# Autodesk Inventor assembly: ROBOT_1_3
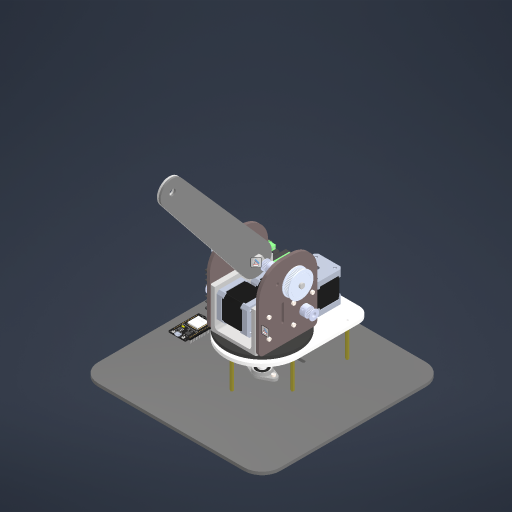
[picture p0: Inventor's stored thumbnail of the model, 512x512]
Saved by Autodesk Inventor 2023 (Build 270158000, 158)
## iProperties
Created: 2023-09-06
Part Number: ROBOT_1_3
Document SubType Name: Assembly
Designer: philo
Sending System: Autodesk Inventor 2023
Preprocessor: ST-DEVELOPER v19
Title: C:\Users\philo\OneDrive\Desktop\HK1-2024\TT ROBOT\3DVer2\ROBOT_1_2.stp
Author: philo
## Documents named in this file (25)
- C:\Users\philo\OneDrive\Desktop\HK1-2024\TT ROBOT\02_3D_design\ROBOT_1_3.iam
- C:\Users\philo\OneDrive\Desktop\HK1-2024\TT ROBOT\02_3D_design\DeRobot.ipt
- C:\Users\philo\OneDrive\Desktop\HK1-2024\TT ROBOT\02_3D_design\Detron.ipt
- C:\Users\philo\OneDrive\Desktop\HK1-2024\TT ROBOT\02_3D_design\goidoObi.ipt
- C:\Users\philo\OneDrive\Desktop\HK1-2024\TT ROBOT\02_3D_design\truday.ipt
- C:\Users\philo\OneDrive\Desktop\HK1-2024\TT ROBOT\02_3D_design\gt2_60teeth.iam
- C:\Users\philo\OneDrive\Desktop\HK1-2024\TT ROBOT\02_3D_design\STEP MOTOR NEMA 17.ipt
- C:\Users\philo\OneDrive\Desktop\HK1-2024\TT ROBOT\02_3D_design\GT2 Pulley 20 Tooth (ID6mm).ipt
- C:\Users\philo\OneDrive\Desktop\HK1-2024\TT ROBOT\02_3D_design\M3 x 5mm.ipt
- C:\Users\philo\OneDrive\Desktop\HK1-2024\TT ROBOT\02_3D_design\Diaquay.ipt
- C:\Users\philo\OneDrive\Desktop\HK1-2024\TT ROBOT\02_3D_design\Tb6600.ipt
- C:\Users\philo\OneDrive\Desktop\HK1-2024\TT ROBOT\02_3D_design\ESP-WROOM32.iam
- C:\Users\philo\OneDrive\Desktop\HK1-2024\TT ROBOT\02_3D_design\codinhtruc.ipt
- C:\Users\philo\OneDrive\Desktop\HK1-2024\TT ROBOT\02_3D_design\daydai.ipt
- C:\Users\philo\OneDrive\Desktop\HK1-2024\TT ROBOT\02_3D_design\gt2smooth.ipt
- C:\Users\philo\OneDrive\Desktop\HK1-2024\TT ROBOT\02_3D_design\trudong5mm.ipt
- C:\Users\philo\OneDrive\Desktop\HK1-2024\TT ROBOT\02_3D_design\trucdogt2.ipt
- C:\Users\philo\OneDrive\Desktop\HK1-2024\TT ROBOT\02_3D_design\HALL.ipt
- C:\Users\philo\OneDrive\Desktop\HK1-2024\TT ROBOT\02_3D_design\namcham.ipt
- C:\Users\philo\OneDrive\Desktop\HK1-2024\TT ROBOT\02_3D_design\Tamop1.ipt
- C:\Users\philo\OneDrive\Desktop\HK1-2024\TT ROBOT\02_3D_design\60pitch pulley GT2 6mm ASSEMBLY.iam
- C:\Users\philo\OneDrive\Desktop\HK1-2024\TT ROBOT\02_3D_design\truc8mm.ipt
- C:\Users\philo\OneDrive\Desktop\HK1-2024\TT ROBOT\02_3D_design\giulink2.ipt
- C:\Users\philo\OneDrive\Documents\Link2Base.ipt
- C:\Users\philo\OneDrive\Desktop\HK1-2024\TT ROBOT\02_3D_design\OcM8.ipt
## Components (61 placed, 24 different names)
1. GT2 Pulley 20 Tooth (ID6mm):4 — Mate:73, Flush:8
2. Link2Base:2 — Mate:74, Mate:75, Mate:76, Mate:78
3. OcM8:1 — Mate:77, Flush:9, Mate:78
4. OcM8:2 — Mate:79, Mate:80
5. DeRobot:1 — Angle:9
6. Detron:1 — Mate:33
7. goidoObi:1
8. goidoObi:2
9. truday:1 — Mate:32
10. gt2_60teeth:1 [sub-assembly]
11. STEP MOTOR NEMA 17:1
12. GT2 Pulley 20 Tooth (ID6mm):1
13. M3 x 5mm:1
14. M3 x 5mm:2
15. M3 x 5mm:3
16. M3 x 5mm:5
17. M3 x 5mm:6
18. M3 x 5mm:7
19. M3 x 5mm:8
20. Tb6600:1
21. Tb6600:2
22. ESP-WROOM32:1 [sub-assembly]
23. daydai:1
24. gt2smooth:1
25. trudong5mm:4
26. trudong5mm:5
27. trudong5mm:6
28. trudong5mm:8
29. trudong5mm:9
30. trucdogt2:1
31. HALL:1
32. M3 x 5mm:9 — Mate:38, Mate:56
33. M3 x 5mm:10 — Mate:39, Mate:58
34. M3 x 5mm:11 — Mate:37, Mate:60
35. M3 x 5mm:12 — Mate:40, Mate:57
36. M3 x 5mm:13 — Mate:41, Mate:61
37. M3 x 5mm:14 — Mate:42, Mate:59
38. M3 x 5mm:15 — Mate:43, Mate:52
39. M3 x 5mm:16 — Mate:45, Mate:51
40. M3 x 5mm:17 — Mate:46, Mate:54
41. M3 x 5mm:18 — Mate:44, Mate:50
42. M3 x 5mm:19 — Mate:47, Mate:53
43. M3 x 5mm:20 — Mate:48, Mate:55
44. gt2smooth:2 — Mate:49
45. giulink2:1 — Mate:63, Angle:3, Angle:4, Angle:5, Angle:6, Angle:7, Angle:8, Mate:64, Mate:65, Mate:67, Flush:4, Flush:5, Mate:68, Mate:69
46. Diaquay:1 — Mate:1, Mate:2, Mate:7, Mate:8, Mate:32, Mate:33, Mate:34, Angle:1, Angle:2, Flush:2, Mate:62, Flush:3, Angle:7
47. codinhtruc:2 — Mate:1, Mate:2, Mate:34, Mate:63
48. namcham:1 — Angle:2, Flush:2, Mate:62, Flush:3
49. STEP MOTOR NEMA 17:2 — Mate:27, Mate:28, Angle:6, Mate:66, Mate:67
50. STEP MOTOR NEMA 17:3 — Mate:26, Mate:30, Angle:5, Angle:8, Mate:64, Mate:65
51. Tamop1:1 — Mate:7, Mate:11, Mate:14, Mate:15, Mate:21, Flush:1, Mate:27, Mate:29, Mate:37, Mate:38, Mate:39, Mate:40, Mate:41, Mate:42, Mate:56, Mate:57, Mate:58, Mate:59, Mate:60, Mate:61, Angle:3, Mate:66, Flush:4, Mate:69, Angle:9
52. goidoObi:3 — Mate:11, Mate:14, Mate:15, Mate:18
53. GT2 Pulley 20 Tooth (ID6mm):2 — Mate:28, Mate:29
54. 60pitch pulley GT2 6mm ASSEMBLY:1 [sub-assembly] — Mate:21, Mate:22
55. Tamop1:2 — Mate:8, Mate:12, Mate:13, Mate:16, Mate:19, Mate:26, Mate:31, Angle:1, Mate:43, Mate:44, Mate:45, Mate:46, Mate:47, Mate:48, Mate:49, Mate:50, Mate:51, Mate:52, Mate:53, Mate:54, Mate:55, Angle:4, Flush:5, Mate:68, Angle:10
56. goidoObi:4 — Mate:12, Mate:13, Mate:16, Mate:17
57. GT2 Pulley 20 Tooth (ID6mm):3 — Mate:30, Mate:31
58. 60pitch pulley GT2 6mm ASSEMBLY:2 [sub-assembly] — Mate:19, Mate:20
59. truc8mm:1 — Mate:18, Mate:22, Mate:23, Flush:1, Mate:73, Flush:8
60. truc8mm:2 — Mate:17, Mate:20, Mate:23, Mate:70, Mate:74, Mate:77, Flush:9, Mate:79
61. Link2Base:1 — Mate:70, Angle:10, Mate:75, Mate:76, Mate:80
## Relationships (85: Mate 68, Angle 10, Flush 7)
- Mate:1: Diaquay:1 ↔ codinhtruc:2
- Mate:2: Diaquay:1 ↔ codinhtruc:2
- Mate:7: Diaquay:1 ↔ Tamop1:1
- Mate:8: Diaquay:1 ↔ Tamop1:2
- Mate:11: Tamop1:1 ↔ goidoObi:3
- Mate:12: Tamop1:2 ↔ goidoObi:4
- Mate:13: Tamop1:2 ↔ goidoObi:4
- Mate:14: Tamop1:1 ↔ goidoObi:3
- Mate:15: Tamop1:1 ↔ goidoObi:3
- Mate:16: Tamop1:2 ↔ goidoObi:4
- Mate:17: goidoObi:4 ↔ truc8mm:2
- Mate:18: goidoObi:3 ↔ truc8mm:1
- Mate:19 (3 mm): Tamop1:2 ↔ 60pitch pulley GT2 6mm ASSEMBLY:2
- Mate:20: 60pitch pulley GT2 6mm ASSEMBLY:2 ↔ truc8mm:2
- Mate:21 (3 mm): Tamop1:1 ↔ 60pitch pulley GT2 6mm ASSEMBLY:1
- Mate:22: 60pitch pulley GT2 6mm ASSEMBLY:1 ↔ truc8mm:1
- Mate:23 (5 mm): truc8mm:1 ↔ truc8mm:2
- Flush:1 (-36 mm): Tamop1:1 ↔ truc8mm:1
- Mate:26: STEP MOTOR NEMA 17:3 ↔ Tamop1:2
- Mate:27: STEP MOTOR NEMA 17:2 ↔ Tamop1:1
- Mate:28: STEP MOTOR NEMA 17:2 ↔ GT2 Pulley 20 Tooth (ID6mm):2
- Mate:29 (3 mm): Tamop1:1 ↔ GT2 Pulley 20 Tooth (ID6mm):2
- Mate:30: STEP MOTOR NEMA 17:3 ↔ GT2 Pulley 20 Tooth (ID6mm):3
- Mate:31 (3 mm): Tamop1:2 ↔ GT2 Pulley 20 Tooth (ID6mm):3
- Mate:32: truday:1 ↔ Diaquay:1
- Mate:33 (6 mm): Detron:1 ↔ Diaquay:1
- Mate:34: Diaquay:1 ↔ codinhtruc:2
- Angle:1 (0 deg): Diaquay:1 ↔ Tamop1:2
- Angle:2 (0 deg): Diaquay:1 ↔ namcham:1
- Flush:2 (-60 mm): Diaquay:1 ↔ namcham:1
- Mate:37: M3 x 5mm:11 ↔ Tamop1:1
- Mate:38: M3 x 5mm:9 ↔ Tamop1:1
- Mate:39: M3 x 5mm:10 ↔ Tamop1:1
- Mate:40: M3 x 5mm:12 ↔ Tamop1:1
- Mate:41: M3 x 5mm:13 ↔ Tamop1:1
- Mate:42: M3 x 5mm:14 ↔ Tamop1:1
- Mate:43: M3 x 5mm:15 ↔ Tamop1:2
- Mate:44: M3 x 5mm:18 ↔ Tamop1:2
- Mate:45: M3 x 5mm:16 ↔ Tamop1:2
- Mate:46: M3 x 5mm:17 ↔ Tamop1:2
- Mate:47: M3 x 5mm:19 ↔ Tamop1:2
- Mate:48: M3 x 5mm:20 ↔ Tamop1:2
- Mate:49 (8 mm): gt2smooth:2 ↔ Tamop1:2
- Mate:50: M3 x 5mm:18 ↔ Tamop1:2
- Mate:51: M3 x 5mm:16 ↔ Tamop1:2
- Mate:52: M3 x 5mm:15 ↔ Tamop1:2
- Mate:53: M3 x 5mm:19 ↔ Tamop1:2
- Mate:54: M3 x 5mm:17 ↔ Tamop1:2
- Mate:55: M3 x 5mm:20 ↔ Tamop1:2
- Mate:56: M3 x 5mm:9 ↔ Tamop1:1
- Mate:57: M3 x 5mm:12 ↔ Tamop1:1
- Mate:58: M3 x 5mm:10 ↔ Tamop1:1
- Mate:59: M3 x 5mm:14 ↔ Tamop1:1
- Mate:60: M3 x 5mm:11 ↔ Tamop1:1
- Mate:61: M3 x 5mm:13 ↔ Tamop1:1
- Mate:62 (-3 mm): Diaquay:1 ↔ namcham:1
- Flush:3: Diaquay:1 ↔ namcham:1
- Mate:63: giulink2:1 ↔ codinhtruc:2
- Angle:3 (90 deg): giulink2:1 ↔ Tamop1:1
- Angle:4 (90 deg): giulink2:1 ↔ Tamop1:2
- Angle:5 (0 deg): giulink2:1 ↔ STEP MOTOR NEMA 17:3
- Angle:6 (0 deg): giulink2:1 ↔ STEP MOTOR NEMA 17:2
- Angle:7 (90 deg): giulink2:1 ↔ Diaquay:1
- Angle:8 (0 deg): giulink2:1 ↔ STEP MOTOR NEMA 17:3
- Mate:64: giulink2:1 ↔ STEP MOTOR NEMA 17:3
- Mate:65: giulink2:1 ↔ STEP MOTOR NEMA 17:3
- Mate:66: STEP MOTOR NEMA 17:2 ↔ Tamop1:1
- Mate:67: giulink2:1 ↔ STEP MOTOR NEMA 17:2
- Flush:4: giulink2:1 ↔ Tamop1:1
- Flush:5: giulink2:1 ↔ Tamop1:2
- Mate:68: giulink2:1 ↔ Tamop1:2
- Mate:69: giulink2:1 ↔ Tamop1:1
- Angle:9 (0 deg): DeRobot:1 ↔ Tamop1:1
- Mate:70: truc8mm:2 ↔ Link2Base:1
- Mate:73: GT2 Pulley 20 Tooth (ID6mm):4 ↔ truc8mm:1
- Flush:8 (3 mm): GT2 Pulley 20 Tooth (ID6mm):4 ↔ truc8mm:1
- Angle:10 (-40 deg): Tamop1:2 ↔ Link2Base:1
- Mate:74: Link2Base:2 ↔ truc8mm:2
- Mate:75: Link2Base:2 ↔ Link2Base:1
- Mate:76: Link2Base:2 ↔ Link2Base:1
- Mate:77: OcM8:1 ↔ truc8mm:2
- Flush:9: OcM8:1 ↔ truc8mm:2
- Mate:78: Link2Base:2 ↔ OcM8:1
- Mate:79: OcM8:2 ↔ truc8mm:2
- Mate:80: OcM8:2 ↔ Link2Base:1
